# Autodesk Inventor assembly: assembly extruder
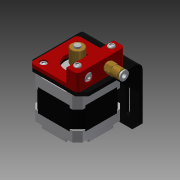
[picture p0: Inventor's stored thumbnail of the model, 180x180]
Saved by Autodesk Inventor 2013 (Build 170138000, 138)
## iProperties
Created: 2015-02-19
Part Number: assembly extruder
Document SubType Name: Assembly
Designer: Noa Izumi
Author: Noa Izumi
## Documents named in this file (9)
- C:\reprap\TinyBoy_v3_20150220\assembly extruder.iam
- C:\reprap\TinyBoy_v3_20150220\stepper_42.iam
- C:\reprap\TinyBoy_v3_20150220\stepper_mount_42.ipt
- C:\reprap\TinyBoy_v3_20150220\extruder_base.ipt
- C:\reprap\TinyBoy_v3_20150220\screw_M3_22_hex.ipt
- C:\reprap\TinyBoy_v3_20150220\screw_M3_10_hex.ipt
- C:\reprap\TinyBoy_v3_20150220\screw_M4_10_hex.ipt
- C:\reprap\TinyBoy_v3_20150220\pc4_m6.ipt
- C:\reprap\TinyBoy_v3_20150220\extruder_gear.ipt
## Components (9 placed, 8 different names)
1. stepper_42:1 [sub-assembly] — 插入:1, 插入:2, 插入:10
2. stepper_mount_42:1 — 插入:1, 插入:2, 插入:3, 插入:4
3. extruder_base:1 — 插入:3, 插入:4, 插入:5, 插入:6, 插入:7, 插入:8, 插入:9, 角度:1
4. screw_M3_22_hex:1 — 插入:6
5. screw_M3_22_hex:2 — 插入:5
6. screw_M3_10_hex:1 — 插入:8
7. screw_M4_10_hex:1 — 插入:7
8. pc4_m6:1 — 插入:9, 角度:1
9. extruder_gear:1 — 插入:10
## Relationships (11: Insert 10, Angle 1)
- 插入:1 [Insert] (0.5 mm): stepper_42:1 ↔ stepper_mount_42:1
- 插入:2 [Insert]: stepper_42:1 ↔ stepper_mount_42:1
- 插入:3 [Insert]: stepper_mount_42:1 ↔ extruder_base:1
- 插入:4 [Insert]: stepper_mount_42:1 ↔ extruder_base:1
- 插入:5 [Insert]: extruder_base:1 ↔ screw_M3_22_hex:2
- 插入:6 [Insert]: extruder_base:1 ↔ screw_M3_22_hex:1
- 插入:7 [Insert]: extruder_base:1 ↔ screw_M4_10_hex:1
- 插入:8 [Insert]: extruder_base:1 ↔ screw_M3_10_hex:1
- 插入:9 [Insert]: extruder_base:1 ↔ pc4_m6:1
- 角度:1 [Angle] (0 deg): extruder_base:1 ↔ pc4_m6:1
- 插入:10 [Insert] (1.5 mm): stepper_42:1 ↔ extruder_gear:1
